# Autodesk Inventor assembly: EL2-C-100
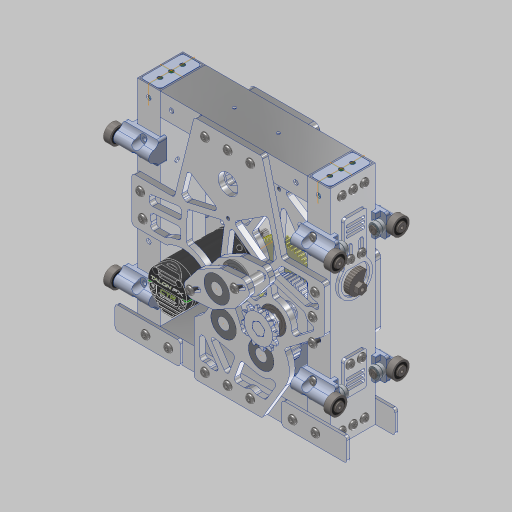
[picture p0: Inventor's stored thumbnail of the model, 512x512]
Saved by Autodesk Inventor 2023.5 (Build 275446000, 446)
## iProperties
Created: 2025-01-11
Part Number: EL2-C-100
Document SubType Name: Assembly
Designer: brand
Mass: 2838.95 g
Surface Area: 6070.12 cm^2
Volume: 958.586 cm^3
Author: brand
## Documents named in this file (14)
- C:\Users\slick\OneDrive\Desktop\2025-ReefScape---CAD\Elevator\EL2\EL2-C-100.iam
- C:\Users\slick\OneDrive\Desktop\2025-ReefScape---CAD\Elevator\EL2\EL2-C-001.ipt
- C:\Users\slick\OneDrive\Desktop\2025-ReefScape---CAD\Elevator\EL2\EL2-005.ipt
- C:\Users\slick\OneDrive\Desktop\2025-ReefScape---CAD\Elevator\EL2\EL2-C-005.ipt
- C:\Users\slick\OneDrive\Desktop\2025-ReefScape---CAD\COMMON PARTS\WCP Elevator parts\WCP-0323\WCP-0323.iam
- C:\Users\slick\OneDrive\Desktop\2025-ReefScape---CAD\Elevator\EL2-CGB\EL2-CGB-100.iam
- C:\Users\slick\OneDrive\Desktop\2025-ReefScape---CAD\Elevator\EL2\EL2-016.ipt
- C:\Users\slick\OneDrive\Desktop\2025-ReefScape---CAD\COMMON PARTS\WCP\WCP-0882.ipt
- C:\Users\slick\OneDrive\Desktop\2025-ReefScape---CAD\Elevator\EL2\EL2-019.ipt
- C:\Users\slick\OneDrive\Desktop\2025-ReefScape---CAD\Elevator\EL2\EL2-C-006.ipt
- C:\Users\slick\OneDrive\Desktop\2025-ReefScape---CAD\STEP files\sen36005_3d_model\sen36005_3d_model.iam
- C:\Users\slick\OneDrive\Desktop\2025-ReefScape---CAD\Content Center\en-US\U UNC 2605\Unbrako - 10 x 1 - 32(10).ipt
- C:\Users\slick\OneDrive\Desktop\2025-ReefScape---CAD\Content Center\en-US\U UNC 2605\Unbrako - 10 x 3_8 - 32(10).ipt
- C:\Users\slick\OneDrive\Desktop\2025-ReefScape---CAD\Content Center\en-US\U UNC 2605\Unbrako - 10 x 1_2 - 32(10).ipt
## Components (91 placed, 13 different names)
1. EL2-C-001:1 — Flush:4, Flush:8, Mate:10, Flush:9, Flush:11, Symmetry:2, Insert:53, Insert:55, Insert:57, Insert:59, Insert:76, Insert:77
2. EL2-C-005:2 — Insert:2, Angle:2, Flush:4, Mate:10, Insert:15, Insert:18, Insert:21, Insert:25, Insert:26, Insert:27, Mate:11, Insert:42, Insert:43, Symmetry:1, Insert:45, Insert:46, Insert:47, Insert:48, Insert:58, Insert:60, Insert:67, Insert:68, Mate:20, Insert:70, Insert:71, Insert:75, Insert:78, Insert:79, Insert:80, Insert:81, Insert:82, Insert:83
3. EL2-C-005:1 — Insert:8, Insert:10, Insert:32, Insert:33, Mate:12, Flush:12, Insert:34, Insert:37, Insert:38, Insert:39, Insert:40, Insert:41, Symmetry:1, Insert:49, Insert:50, Insert:54, Insert:56, Mate:19, Insert:65, Insert:66, Mate:21, Insert:72, Insert:73, Insert:74, Insert:84, Insert:85, Insert:86, Insert:87, Insert:88, Insert:89
4. EL2-C-001:4 — Flush:10, Flush:11, Mate:11, Mate:12, Flush:12, Symmetry:2, Insert:51, Insert:52
5. EL2-005:1 — Insert:2, Angle:2, Flush:9
6. EL2-005:2 — Insert:8, Flush:8
7. EL2-005:3 — Insert:10, Flush:10, Insert:32, Insert:33
8. EL2-005:4 — Insert:42, Insert:43
9. WCP-0323:1 [sub-assembly] — Insert:34, Insert:49, Insert:100
10. WCP-0323:2 [sub-assembly] — Insert:40, Insert:41
11. WCP-0323:3 [sub-assembly] — Insert:38, Insert:39, Insert:131
12. WCP-0323:4 [sub-assembly] — Insert:25, Insert:27, Insert:46, Insert:98
13. WCP-0323:5 [sub-assembly] — Insert:18, Insert:26, Insert:130
14. WCP-0323:6 [sub-assembly] — Insert:15, Insert:48, Insert:102
15. WCP-0323:7 [sub-assembly] — Insert:21, Insert:45, Insert:47, Insert:99
16. WCP-0323:8 [sub-assembly] — Insert:37, Insert:50, Insert:101
17. EL2-CGB-100:1 [sub-assembly] — Insert:51, Insert:52, Mate:22, Mate:23, Mate:48, Mate:49, Mate:50, Mate:51, Mate:52, Mate:53, Mate:54, Mate:55, Mate:56, Mate:57, Mate:58, Mate:59, Mate:60, Mate:61, Mate:62, Mate:63, Mate:64, Mate:65, Mate:66, Mate:67, Mate:68, Mate:69, Insert:103, Insert:105, Insert:106, Insert:115, Insert:116, Insert:117, Insert:118, Insert:119, Insert:120, Insert:121, Insert:122, Insert:123, Insert:124, Insert:125, Insert:126, Insert:129
18. EL2-016:1 — Insert:53, Insert:54, Insert:107, Insert:113
19. EL2-016:2 — Insert:55, Insert:56, Insert:110, Insert:112
20. EL2-016:3 — Insert:57, Insert:58, Insert:109, Insert:111
21. EL2-016:4 — Insert:59, Insert:60, Insert:108, Insert:114
22. WCP-0882:1 — Insert:75
23. WCP-0882:2 — Insert:74
24. EL2-019:1 — Mate:19, Insert:65, Insert:66, Insert:92, Insert:93
25. EL2-019:2 — Insert:67, Insert:68, Insert:94, Insert:95
26. EL2-C-006:1 — Mate:20, Insert:70, Insert:71, Insert:96, Insert:97
27. EL2-C-006:2 — Mate:21, Insert:72, Insert:73, Insert:90, Insert:91
28. sen36005_3d_model:1 [sub-assembly] — Insert:76, Insert:77
29. Unbrako UNC Hex Socket Button Cap - Inch 10 x 1:1 — Mate:22, Mate:23
30. Unbrako UNC Hex Socket Button Cap - Inch 10 x 1:14 — Mate:48, Mate:49
31. Unbrako UNC Hex Socket Button Cap - Inch 10 x 1:15 — Mate:50, Mate:51
32. Unbrako UNC Hex Socket Button Cap - Inch 10 x 1:16 — Mate:52, Mate:53
33. Unbrako UNC Hex Socket Button Cap - Inch 10 x 1:17 — Mate:54, Mate:55
34. Unbrako UNC Hex Socket Button Cap - Inch 10 x 1:18 — Mate:56, Mate:57
35. Unbrako UNC Hex Socket Button Cap - Inch 10 x 1:19 — Mate:58, Mate:59
36. Unbrako UNC Hex Socket Button Cap - Inch 10 x 1:20 — Mate:60, Mate:61
37. Unbrako UNC Hex Socket Button Cap - Inch 10 x 1:21 — Mate:62, Mate:63
38. Unbrako UNC Hex Socket Button Cap - Inch 10 x 1:22 — Mate:64, Mate:65
39. Unbrako UNC Hex Socket Button Cap - Inch 10 x 1:23 — Mate:66, Mate:67
40. Unbrako UNC Hex Socket Button Cap - Inch 10 x 1:24 — Mate:68, Mate:69
41. Unbrako UNC Hex Socket Button Cap - Inch 10 x 3/8:1 — Insert:78
42. Unbrako UNC Hex Socket Button Cap - Inch 10 x 3/8:2 — Insert:79
43. Unbrako UNC Hex Socket Button Cap - Inch 10 x 3/8:3 — Insert:80
44. Unbrako UNC Hex Socket Button Cap - Inch 10 x 3/8:4 — Insert:81
45. Unbrako UNC Hex Socket Button Cap - Inch 10 x 3/8:5 — Insert:82
46. Unbrako UNC Hex Socket Button Cap - Inch 10 x 3/8:6 — Insert:83
47. Unbrako UNC Hex Socket Button Cap - Inch 10 x 3/8:7 — Insert:84
48. Unbrako UNC Hex Socket Button Cap - Inch 10 x 3/8:8 — Insert:85
49. Unbrako UNC Hex Socket Button Cap - Inch 10 x 3/8:9 — Insert:86
50. Unbrako UNC Hex Socket Button Cap - Inch 10 x 3/8:10 — Insert:87
51. Unbrako UNC Hex Socket Button Cap - Inch 10 x 3/8:11 — Insert:88
52. Unbrako UNC Hex Socket Button Cap - Inch 10 x 3/8:12 — Insert:89
53. Unbrako UNC Hex Socket Button Cap - Inch 10 x 1:25 — Insert:90
54. Unbrako UNC Hex Socket Button Cap - Inch 10 x 1:26 — Insert:91
55. Unbrako UNC Hex Socket Button Cap - Inch 10 x 1:27 — Insert:92
56. Unbrako UNC Hex Socket Button Cap - Inch 10 x 1:28 — Insert:93
57. Unbrako UNC Hex Socket Button Cap - Inch 10 x 1:29 — Insert:94
58. Unbrako UNC Hex Socket Button Cap - Inch 10 x 1:30 — Insert:95
59. Unbrako UNC Hex Socket Button Cap - Inch 10 x 1:31 — Insert:96
60. Unbrako UNC Hex Socket Button Cap - Inch 10 x 1:32 — Insert:97
61. Unbrako UNC Hex Socket Button Cap - Inch 10 x 1:33 — Insert:98
62. Unbrako UNC Hex Socket Button Cap - Inch 10 x 1:34 — Insert:99
63. Unbrako UNC Hex Socket Button Cap - Inch 10 x 1:35 — Insert:100
64. Unbrako UNC Hex Socket Button Cap - Inch 10 x 1:36 — Insert:101
65. Unbrako UNC Hex Socket Button Cap - Inch 10 x 1:37 — Insert:102
66. Unbrako UNC Hex Socket Button Cap - Inch 10 x 3/8:13 — Insert:103
67. Unbrako UNC Hex Socket Button Cap - Inch 10 x 3/8:15 — Insert:105
68. Unbrako UNC Hex Socket Button Cap - Inch 10 x 3/8:16 — Insert:106
69. Unbrako UNC Hex Socket Button Cap - Inch 10 x 1/2:1 — Insert:107
70. Unbrako UNC Hex Socket Button Cap - Inch 10 x 1/2:2 — Insert:108
71. Unbrako UNC Hex Socket Button Cap - Inch 10 x 1/2:3 — Insert:109
72. Unbrako UNC Hex Socket Button Cap - Inch 10 x 1/2:4 — Insert:110
73. Unbrako UNC Hex Socket Button Cap - Inch 10 x 1:38 — Insert:111
74. Unbrako UNC Hex Socket Button Cap - Inch 10 x 1:39 — Insert:112
75. Unbrako UNC Hex Socket Button Cap - Inch 10 x 1:40 — Insert:113
76. Unbrako UNC Hex Socket Button Cap - Inch 10 x 1:41 — Insert:114
77. Unbrako UNC Hex Socket Button Cap - Inch 10 x 1:42 — Insert:115
78. Unbrako UNC Hex Socket Button Cap - Inch 10 x 1:43 — Insert:116
79. Unbrako UNC Hex Socket Button Cap - Inch 10 x 1:44 — Insert:117
80. Unbrako UNC Hex Socket Button Cap - Inch 10 x 1:45 — Insert:118
81. Unbrako UNC Hex Socket Button Cap - Inch 10 x 1:46 — Insert:119
82. Unbrako UNC Hex Socket Button Cap - Inch 10 x 1:47 — Insert:120
83. Unbrako UNC Hex Socket Button Cap - Inch 10 x 1:48 — Insert:121
84. Unbrako UNC Hex Socket Button Cap - Inch 10 x 1:49 — Insert:122
85. Unbrako UNC Hex Socket Button Cap - Inch 10 x 1:50 — Insert:123
86. Unbrako UNC Hex Socket Button Cap - Inch 10 x 1:51 — Insert:124
87. Unbrako UNC Hex Socket Button Cap - Inch 10 x 1:52 — Insert:125
88. Unbrako UNC Hex Socket Button Cap - Inch 10 x 1:53 — Insert:126
89. Unbrako UNC Hex Socket Button Cap - Inch 10 x 1:56 — Insert:129
90. Unbrako UNC Hex Socket Button Cap - Inch 10 x 1:57 — Insert:130
91. Unbrako UNC Hex Socket Button Cap - Inch 10 x 1:58 — Insert:131
## Relationships (139: Insert 98, Mate 32, Flush 6, Symmetry 2, Angle 1)
- Insert:2: EL2-C-005:2 ↔ EL2-005:1
- Angle:2 (0 deg): EL2-C-005:2 ↔ EL2-005:1
- Insert:8: EL2-C-005:1 ↔ EL2-005:2
- Insert:10: EL2-C-005:1 ↔ EL2-005:3
- Flush:4: EL2-C-001:1 ↔ EL2-C-005:2
- Flush:8: EL2-C-001:1 ↔ EL2-005:2
- Mate:10: EL2-C-001:1 ↔ EL2-C-005:2
- Flush:9: EL2-C-001:1 ↔ EL2-005:1
- Flush:10: EL2-C-001:4 ↔ EL2-005:3
- Flush:11: EL2-C-001:1 ↔ EL2-C-001:4
- Insert:15: EL2-C-005:2 ↔ WCP-0323:6
- Insert:18: EL2-C-005:2 ↔ WCP-0323:5
- Insert:21: EL2-C-005:2 ↔ WCP-0323:7
- Insert:25: EL2-C-005:2 ↔ WCP-0323:4
- Insert:26: EL2-C-005:2 ↔ WCP-0323:5
- Insert:27: EL2-C-005:2 ↔ WCP-0323:4
- Insert:32: EL2-C-005:1 ↔ EL2-005:3
- Insert:33: EL2-C-005:1 ↔ EL2-005:3
- Mate:11: EL2-C-005:2 ↔ EL2-C-001:4
- Mate:12: EL2-C-005:1 ↔ EL2-C-001:4
- Flush:12: EL2-C-005:1 ↔ EL2-C-001:4
- Insert:34: EL2-C-005:1 ↔ WCP-0323:1
- Insert:37: EL2-C-005:1 ↔ WCP-0323:8
- Insert:38: EL2-C-005:1 ↔ WCP-0323:3
- Insert:39: EL2-C-005:1 ↔ WCP-0323:3
- Insert:40: EL2-C-005:1 ↔ WCP-0323:2
- Insert:41: EL2-C-005:1 ↔ WCP-0323:2
- Insert:42: EL2-C-005:2 ↔ EL2-005:4
- Insert:43: EL2-C-005:2 ↔ EL2-005:4
- Symmetry:1: EL2-C-005:2 ↔ EL2-C-005:1
- Symmetry:2: EL2-C-001:1 ↔ EL2-C-001:4
- Mate:13
- Mate:14
- Insert:45: EL2-C-005:2 ↔ WCP-0323:7
- Insert:46: EL2-C-005:2 ↔ WCP-0323:4
- Insert:47: EL2-C-005:2 ↔ WCP-0323:7
- Insert:48: EL2-C-005:2 ↔ WCP-0323:6
- Insert:49: EL2-C-005:1 ↔ WCP-0323:1
- Insert:50: EL2-C-005:1 ↔ WCP-0323:8
- Insert:51: EL2-C-001:4 ↔ EL2-CGB-100:1
- Insert:52: EL2-C-001:4 ↔ EL2-CGB-100:1
- Insert:53: EL2-C-001:1 ↔ EL2-016:1
- Insert:54: EL2-C-005:1 ↔ EL2-016:1
- Insert:55: EL2-C-001:1 ↔ EL2-016:2
- Insert:56: EL2-C-005:1 ↔ EL2-016:2
- Insert:57: EL2-C-001:1 ↔ EL2-016:3
- Insert:58: EL2-C-005:2 ↔ EL2-016:3
- Insert:59: EL2-C-001:1 ↔ EL2-016:4
- Insert:60: EL2-C-005:2 ↔ EL2-016:4
- Mate:19: EL2-C-005:1 ↔ EL2-019:1
- Insert:65: EL2-C-005:1 ↔ EL2-019:1
- Insert:66: EL2-C-005:1 ↔ EL2-019:1
- Insert:67: EL2-C-005:2 ↔ EL2-019:2
- Insert:68: EL2-C-005:2 ↔ EL2-019:2
- Mate:20: EL2-C-005:2 ↔ EL2-C-006:1
- Insert:70: EL2-C-005:2 ↔ EL2-C-006:1
- Insert:71: EL2-C-005:2 ↔ EL2-C-006:1
- Mate:21: EL2-C-005:1 ↔ EL2-C-006:2
- Insert:72: EL2-C-005:1 ↔ EL2-C-006:2
- Insert:73: EL2-C-005:1 ↔ EL2-C-006:2
- Insert:74: EL2-C-005:1 ↔ WCP-0882:2
- Insert:75: EL2-C-005:2 ↔ WCP-0882:1
- Insert:76: EL2-C-001:1 ↔ sen36005_3d_model:1
- Insert:77: EL2-C-001:1 ↔ sen36005_3d_model:1
- Mate:22: EL2-CGB-100:1 ↔ Unbrako UNC Hex Socket Button Cap - Inch 10 x 1:1
- Mate:23: EL2-CGB-100:1 ↔ Unbrako UNC Hex Socket Button Cap - Inch 10 x 1:1
- Mate:48: EL2-CGB-100:1 ↔ Unbrako UNC Hex Socket Button Cap - Inch 10 x 1:14
- Mate:49: EL2-CGB-100:1 ↔ Unbrako UNC Hex Socket Button Cap - Inch 10 x 1:14
- Mate:50: EL2-CGB-100:1 ↔ Unbrako UNC Hex Socket Button Cap - Inch 10 x 1:15
- Mate:51: EL2-CGB-100:1 ↔ Unbrako UNC Hex Socket Button Cap - Inch 10 x 1:15
- Mate:52: EL2-CGB-100:1 ↔ Unbrako UNC Hex Socket Button Cap - Inch 10 x 1:16
- Mate:53: EL2-CGB-100:1 ↔ Unbrako UNC Hex Socket Button Cap - Inch 10 x 1:16
- Mate:54: EL2-CGB-100:1 ↔ Unbrako UNC Hex Socket Button Cap - Inch 10 x 1:17
- Mate:55: EL2-CGB-100:1 ↔ Unbrako UNC Hex Socket Button Cap - Inch 10 x 1:17
- Mate:56: EL2-CGB-100:1 ↔ Unbrako UNC Hex Socket Button Cap - Inch 10 x 1:18
- Mate:57: EL2-CGB-100:1 ↔ Unbrako UNC Hex Socket Button Cap - Inch 10 x 1:18
- Mate:58: EL2-CGB-100:1 ↔ Unbrako UNC Hex Socket Button Cap - Inch 10 x 1:19
- Mate:59: EL2-CGB-100:1 ↔ Unbrako UNC Hex Socket Button Cap - Inch 10 x 1:19
- Mate:60: EL2-CGB-100:1 ↔ Unbrako UNC Hex Socket Button Cap - Inch 10 x 1:20
- Mate:61: EL2-CGB-100:1 ↔ Unbrako UNC Hex Socket Button Cap - Inch 10 x 1:20
- Mate:62: EL2-CGB-100:1 ↔ Unbrako UNC Hex Socket Button Cap - Inch 10 x 1:21
- Mate:63: EL2-CGB-100:1 ↔ Unbrako UNC Hex Socket Button Cap - Inch 10 x 1:21
- Mate:64: EL2-CGB-100:1 ↔ Unbrako UNC Hex Socket Button Cap - Inch 10 x 1:22
- Mate:65: EL2-CGB-100:1 ↔ Unbrako UNC Hex Socket Button Cap - Inch 10 x 1:22
- Mate:66: EL2-CGB-100:1 ↔ Unbrako UNC Hex Socket Button Cap - Inch 10 x 1:23
- Mate:67: EL2-CGB-100:1 ↔ Unbrako UNC Hex Socket Button Cap - Inch 10 x 1:23
- Mate:68: EL2-CGB-100:1 ↔ Unbrako UNC Hex Socket Button Cap - Inch 10 x 1:24
- Mate:69: EL2-CGB-100:1 ↔ Unbrako UNC Hex Socket Button Cap - Inch 10 x 1:24
- Insert:78: EL2-C-005:2 ↔ Unbrako UNC Hex Socket Button Cap - Inch 10 x 3/8:1
- Insert:79: EL2-C-005:2 ↔ Unbrako UNC Hex Socket Button Cap - Inch 10 x 3/8:2
- Insert:80: EL2-C-005:2 ↔ Unbrako UNC Hex Socket Button Cap - Inch 10 x 3/8:3
- Insert:81: EL2-C-005:2 ↔ Unbrako UNC Hex Socket Button Cap - Inch 10 x 3/8:4
- Insert:82: EL2-C-005:2 ↔ Unbrako UNC Hex Socket Button Cap - Inch 10 x 3/8:5
- Insert:83: EL2-C-005:2 ↔ Unbrako UNC Hex Socket Button Cap - Inch 10 x 3/8:6
- Insert:84: EL2-C-005:1 ↔ Unbrako UNC Hex Socket Button Cap - Inch 10 x 3/8:7
- Insert:85: EL2-C-005:1 ↔ Unbrako UNC Hex Socket Button Cap - Inch 10 x 3/8:8
- Insert:86: EL2-C-005:1 ↔ Unbrako UNC Hex Socket Button Cap - Inch 10 x 3/8:9
- Insert:87: EL2-C-005:1 ↔ Unbrako UNC Hex Socket Button Cap - Inch 10 x 3/8:10
- Insert:88: EL2-C-005:1 ↔ Unbrako UNC Hex Socket Button Cap - Inch 10 x 3/8:11
- Insert:89: EL2-C-005:1 ↔ Unbrako UNC Hex Socket Button Cap - Inch 10 x 3/8:12
- Insert:90: EL2-C-006:2 ↔ Unbrako UNC Hex Socket Button Cap - Inch 10 x 1:25
- Insert:91: EL2-C-006:2 ↔ Unbrako UNC Hex Socket Button Cap - Inch 10 x 1:26
- Insert:92: EL2-019:1 ↔ Unbrako UNC Hex Socket Button Cap - Inch 10 x 1:27
- Insert:93: EL2-019:1 ↔ Unbrako UNC Hex Socket Button Cap - Inch 10 x 1:28
- Insert:94: EL2-019:2 ↔ Unbrako UNC Hex Socket Button Cap - Inch 10 x 1:29
- Insert:95: EL2-019:2 ↔ Unbrako UNC Hex Socket Button Cap - Inch 10 x 1:30
- Insert:96: EL2-C-006:1 ↔ Unbrako UNC Hex Socket Button Cap - Inch 10 x 1:31
- Insert:97: EL2-C-006:1 ↔ Unbrako UNC Hex Socket Button Cap - Inch 10 x 1:32
- Insert:98: WCP-0323:4 ↔ Unbrako UNC Hex Socket Button Cap - Inch 10 x 1:33
- Insert:99: WCP-0323:7 ↔ Unbrako UNC Hex Socket Button Cap - Inch 10 x 1:34
- Insert:100: WCP-0323:1 ↔ Unbrako UNC Hex Socket Button Cap - Inch 10 x 1:35
- Insert:101: WCP-0323:8 ↔ Unbrako UNC Hex Socket Button Cap - Inch 10 x 1:36
- Insert:102: WCP-0323:6 ↔ Unbrako UNC Hex Socket Button Cap - Inch 10 x 1:37
- Insert:103: EL2-CGB-100:1 ↔ Unbrako UNC Hex Socket Button Cap - Inch 10 x 3/8:13
- Insert:105: EL2-CGB-100:1 ↔ Unbrako UNC Hex Socket Button Cap - Inch 10 x 3/8:15
- Insert:106: EL2-CGB-100:1 ↔ Unbrako UNC Hex Socket Button Cap - Inch 10 x 3/8:16
- Insert:107: EL2-016:1 ↔ Unbrako UNC Hex Socket Button Cap - Inch 10 x 1/2:1
- Insert:108: EL2-016:4 ↔ Unbrako UNC Hex Socket Button Cap - Inch 10 x 1/2:2
- Insert:109: EL2-016:3 ↔ Unbrako UNC Hex Socket Button Cap - Inch 10 x 1/2:3
- Insert:110: EL2-016:2 ↔ Unbrako UNC Hex Socket Button Cap - Inch 10 x 1/2:4
- Insert:111: EL2-016:3 ↔ Unbrako UNC Hex Socket Button Cap - Inch 10 x 1:38
- Insert:112: EL2-016:2 ↔ Unbrako UNC Hex Socket Button Cap - Inch 10 x 1:39
- Insert:113: EL2-016:1 ↔ Unbrako UNC Hex Socket Button Cap - Inch 10 x 1:40
- Insert:114: EL2-016:4 ↔ Unbrako UNC Hex Socket Button Cap - Inch 10 x 1:41
- Insert:115: EL2-CGB-100:1 ↔ Unbrako UNC Hex Socket Button Cap - Inch 10 x 1:42
- Insert:116: EL2-CGB-100:1 ↔ Unbrako UNC Hex Socket Button Cap - Inch 10 x 1:43
- Insert:117: EL2-CGB-100:1 ↔ Unbrako UNC Hex Socket Button Cap - Inch 10 x 1:44
- Insert:118: EL2-CGB-100:1 ↔ Unbrako UNC Hex Socket Button Cap - Inch 10 x 1:45
- Insert:119: EL2-CGB-100:1 ↔ Unbrako UNC Hex Socket Button Cap - Inch 10 x 1:46
- Insert:120: EL2-CGB-100:1 ↔ Unbrako UNC Hex Socket Button Cap - Inch 10 x 1:47
- Insert:121: EL2-CGB-100:1 ↔ Unbrako UNC Hex Socket Button Cap - Inch 10 x 1:48
- Insert:122: EL2-CGB-100:1 ↔ Unbrako UNC Hex Socket Button Cap - Inch 10 x 1:49
- Insert:123: EL2-CGB-100:1 ↔ Unbrako UNC Hex Socket Button Cap - Inch 10 x 1:50
- Insert:124: EL2-CGB-100:1 ↔ Unbrako UNC Hex Socket Button Cap - Inch 10 x 1:51
- Insert:125: EL2-CGB-100:1 ↔ Unbrako UNC Hex Socket Button Cap - Inch 10 x 1:52
- Insert:126: EL2-CGB-100:1 ↔ Unbrako UNC Hex Socket Button Cap - Inch 10 x 1:53
- Insert:129: EL2-CGB-100:1 ↔ Unbrako UNC Hex Socket Button Cap - Inch 10 x 1:56
- Insert:130: WCP-0323:5 ↔ Unbrako UNC Hex Socket Button Cap - Inch 10 x 1:57
- Insert:131: WCP-0323:3 ↔ Unbrako UNC Hex Socket Button Cap - Inch 10 x 1:58
